# Autodesk Inventor assembly: Link3
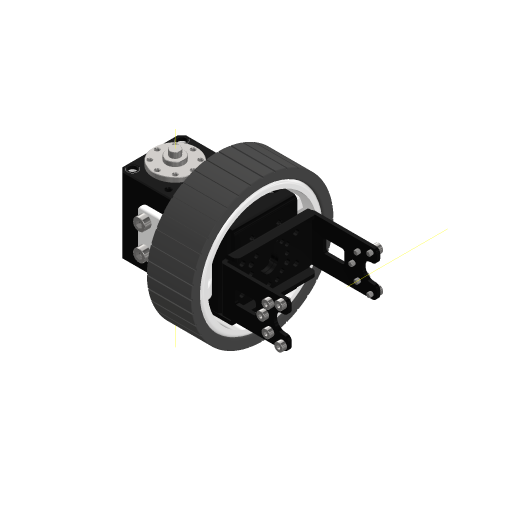
[picture p0: Inventor's stored thumbnail of the model, 512x512]
Saved by Autodesk Inventor 2024 (Build 280153000, 153)
## iProperties
Created: 2022-11-03
Part Number: Link3
Document SubType Name: Assembly
Designer: doore
Mass: 123.815 g
Surface Area: 411.684 cm^2
Volume: 81.3149 cm^3
Density: 1.52266 g/cm^3
Author: doore
## Documents named in this file (5)
- C:\Users\Bong\project\snake_RL\matlab\meshes\Inventor_Reallign\linkB\LinkB.iam
- C:\Users\Bong\project\snake_RL\matlab\meshes\Inventor_Reallign\linkB\Haed.iam
- C:\Users\Bong\project\snake_RL\matlab\meshes\Inventor_Reallign\linkB\xm430_frame.ipt
- C:\Users\Bong\project\snake_RL\matlab\meshes\Inventor_Reallign\linkB\xm430_hinge.ipt
- C:\Users\Bong\Documents\Inventor\Content Center Files\R2024\ko-KR\BS 4168(1)\BS 4168 - M2 x 3(1).ipt
## Components (13 placed, 4 different names)
1. Haed:1 [sub-assembly] — 강체:1, 메이트:3, 메이트:4
2. xm430_frame:1 — 강체:1, 강체:2
3. xm430_hinge:1 — 강체:2, 강체:3, 강체:4, 강체:5, 강체:6, 강체:7, 강체:8, 강체:9, 강체:10, 강체:11, 강체:12, 메이트:1
4. BS 4168 : 부품 1 6각 소켓 머리 캡 나사 - 미터 M2 x 3:1 — 강체:4
5. BS 4168 : 부품 1 6각 소켓 머리 캡 나사 - 미터 M2 x 3:2 — 강체:7
6. BS 4168 : 부품 1 6각 소켓 머리 캡 나사 - 미터 M2 x 3:3 — 강체:6
7. BS 4168 : 부품 1 6각 소켓 머리 캡 나사 - 미터 M2 x 3:4 — 강체:5
8. BS 4168 : 부품 1 6각 소켓 머리 캡 나사 - 미터 M2 x 3:5 — 강체:3
9. BS 4168 : 부품 1 6각 소켓 머리 캡 나사 - 미터 M2 x 3:6 — 강체:9
10. BS 4168 : 부품 1 6각 소켓 머리 캡 나사 - 미터 M2 x 3:7 — 강체:11
11. BS 4168 : 부품 1 6각 소켓 머리 캡 나사 - 미터 M2 x 3:8 — 강체:8
12. BS 4168 : 부품 1 6각 소켓 머리 캡 나사 - 미터 M2 x 3:9 — 강체:10
13. BS 4168 : 부품 1 6각 소켓 머리 캡 나사 - 미터 M2 x 3:10 — 강체:12
## Relationships (16: WeldJoint 12, Mate 4)
- 강체:1 [WeldJoint]: Haed:1 ↔ xm430_frame:1
- 강체:2 [WeldJoint]: xm430_frame:1 ↔ xm430_hinge:1
- 강체:3 [WeldJoint]: xm430_hinge:1 ↔ BS 4168 : 부품 1 6각 소켓 머리 캡 나사 - 미터 M2 x 3:5
- 강체:4 [WeldJoint]: xm430_hinge:1 ↔ BS 4168 : 부품 1 6각 소켓 머리 캡 나사 - 미터 M2 x 3:1
- 강체:5 [WeldJoint]: xm430_hinge:1 ↔ BS 4168 : 부품 1 6각 소켓 머리 캡 나사 - 미터 M2 x 3:4
- 강체:6 [WeldJoint]: xm430_hinge:1 ↔ BS 4168 : 부품 1 6각 소켓 머리 캡 나사 - 미터 M2 x 3:3
- 강체:7 [WeldJoint]: xm430_hinge:1 ↔ BS 4168 : 부품 1 6각 소켓 머리 캡 나사 - 미터 M2 x 3:2
- 강체:8 [WeldJoint]: xm430_hinge:1 ↔ BS 4168 : 부품 1 6각 소켓 머리 캡 나사 - 미터 M2 x 3:8
- 강체:9 [WeldJoint]: xm430_hinge:1 ↔ BS 4168 : 부품 1 6각 소켓 머리 캡 나사 - 미터 M2 x 3:6
- 강체:10 [WeldJoint]: xm430_hinge:1 ↔ BS 4168 : 부품 1 6각 소켓 머리 캡 나사 - 미터 M2 x 3:9
- 강체:11 [WeldJoint]: xm430_hinge:1 ↔ BS 4168 : 부품 1 6각 소켓 머리 캡 나사 - 미터 M2 x 3:7
- 강체:12 [WeldJoint]: xm430_hinge:1 ↔ BS 4168 : 부품 1 6각 소켓 머리 캡 나사 - 미터 M2 x 3:10
- 메이트:1 [Mate]: xm430_hinge:1
- 메이트:2 [Mate]
- 메이트:3 [Mate]: Haed:1
- 메이트:4 [Mate]: Haed:1
